# Autodesk Inventor assembly: STLassem
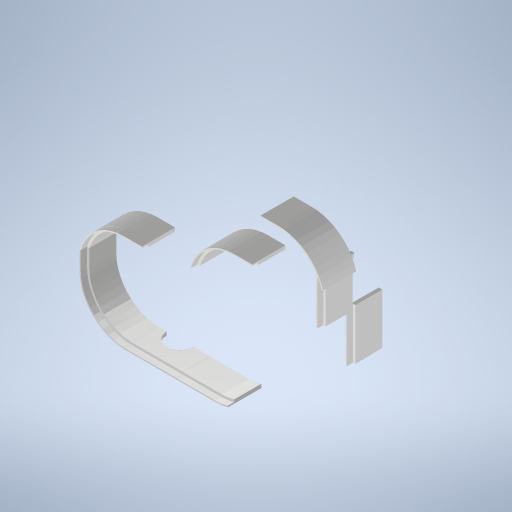
[picture p0: Inventor's stored thumbnail of the model, 512x512]
Saved by Autodesk Inventor 2024 (Build 280153000, 153)
## iProperties
Created: 2024-01-03
Part Number: STLassem
Document SubType Name: Assembly
Designer: Brian
Author: Brian
## Documents named in this file (9)
- C:\Users\brian\OneDrive\Documents\Inventor\drinkSilo\STLassem.iam
- C:\Users\brian\OneDrive\Documents\Inventor\drinkSilo\cutSTLs\B1.ipt
- C:\Users\brian\OneDrive\Documents\Inventor\drinkSilo\cutSTLs\B2.ipt
- C:\Users\brian\OneDrive\Documents\Inventor\drinkSilo\cutSTLs\B3.ipt
- C:\Users\brian\OneDrive\Documents\Inventor\drinkSilo\cutSTLs\B4.ipt
- C:\Users\brian\OneDrive\Documents\Inventor\drinkSilo\cutSTLs\B5.ipt
- C:\Users\brian\OneDrive\Documents\Inventor\drinkSilo\cutSTLs\B6.ipt
- C:\Users\brian\OneDrive\Documents\Inventor\drinkSilo\cutSTLs\B7.ipt
- C:\Users\brian\OneDrive\Documents\Inventor\drinkSilo\cutSTLs\B8.ipt
## Components (8 placed, 8 different names)
1. B1:1 — Mate:1, Flush:1, Mate:2
2. B2:2
3. B3:1 — Mate:1, Flush:1, Mate:2, Flush:2, Mate:3, Mate:4
4. B4:1 — Flush:2, Mate:3, Mate:4, Flush:3, Mate:5
5. B5:1
6. B6:1
7. B7:1 — Flush:3, Mate:5
8. B8:1
## Relationships (8: Mate 5, Flush 3)
- Mate:1: B1:1 ↔ B3:1
- Flush:1: B1:1 ↔ B3:1
- Mate:2: B1:1 ↔ B3:1
- Flush:2: B3:1 ↔ B4:1
- Mate:3: B3:1 ↔ B4:1
- Mate:4: B3:1 ↔ B4:1
- Flush:3: B4:1 ↔ B7:1
- Mate:5: B4:1 ↔ B7:1
